# Autodesk Inventor assembly: Ring
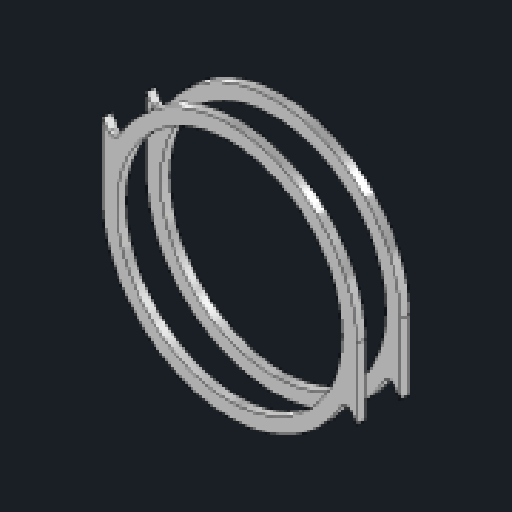
[picture p0: Inventor's stored thumbnail of the model, 512x512]
Saved by Autodesk Inventor 2023.2 (Build 272271030, 271C)
## iProperties
Created: 2024-03-01
Part Number: Ring
Document SubType Name: Assembly
Designer: robpl
Author: robpl
## Documents named in this file (2)
- C:\Users\robpl\OneDrive\Documents\Arduino\Onslaught\CAD\Onslaught V2\Ring.iam
- C:\Users\robpl\OneDrive\Documents\Arduino\Onslaught\CAD\Onslaught V2\Weapon.ipt
## Components (2 placed, 1 different names)
1. Weapon:1 — Mate:1, Mate:2, Mate:3
2. Weapon:2 — Mate:1, Mate:2, Mate:3
## Relationships (3: Mate 3)
- Mate:1: Weapon:1 ↔ Weapon:2
- Mate:2: Weapon:1 ↔ Weapon:2
- Mate:3 (-29.6 mm): Weapon:1 ↔ Weapon:2
